# Autodesk Inventor assembly: ASY Beshkino_bio_tank
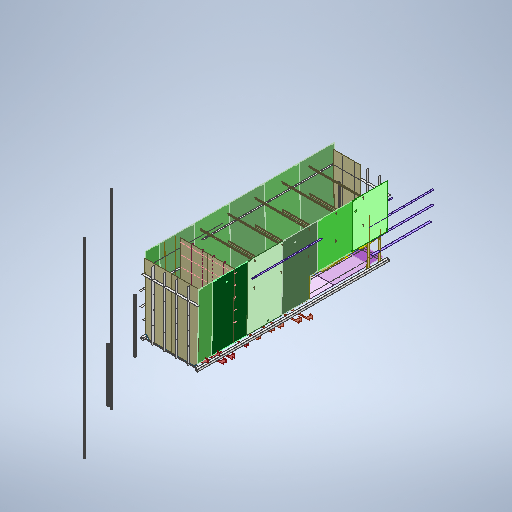
[picture p0: Inventor's stored thumbnail of the model, 512x512]
Saved by Autodesk Inventor 2025 (Build 290162010, 162A)
## iProperties
Created: 2024-07-21
Part Number: ASY Beshkino_bio_tank
Document SubType Name: Assembly
Designer: admin
Mass: 5.81287e+06 g
Surface Area: 2.77755e+06 cm^2
Volume: 3.12018e+06 cm^3
Density: 1.86299 g/cm^3
Author: admin
## Documents named in this file (40)
- C:\Users\pokla\Documents\Inventor\BSH_Beshkino_bio_tank\ASY Beshkino_bio_tank.iam
- C:\Users\pokla\Documents\Inventor\BSH_Beshkino_bio_tank\BSH 000 dim Beshkino_bio_tank.ipt
- C:\Users\pokla\Documents\Inventor\BSH_Beshkino_bio_tank\BSH 011 floor.ipt
- C:\Users\pokla\Documents\Inventor\BSH_Beshkino_bio_tank\BSH 021 rib floor.ipt
- C:\Users\pokla\Documents\Inventor\BSH_Beshkino_bio_tank\BSH 022 rib board.ipt
- C:\Users\pokla\Documents\Inventor\BSH_Beshkino_bio_tank\BSH 076 tube.ipt
- C:\Users\pokla\Documents\Inventor\BSH_Beshkino_bio_tank\BSH 061 butt end.ipt
- C:\Users\pokla\Documents\Inventor\BSH_Beshkino_bio_tank\BSH 041 board.ipt
- C:\Users\pokla\Documents\Inventor\BSH_Beshkino_bio_tank\BSH 047 board.ipt
- C:\Users\pokla\Documents\Inventor\BSH_Beshkino_bio_tank\BSH 033 stringer board 1.ipt
- C:\Users\pokla\Documents\Inventor\BSH_Beshkino_bio_tank\BSH 045 back.ipt
- C:\Users\pokla\Documents\Inventor\BSH_Beshkino_bio_tank\BSH 031 stringer floor.ipt
- C:\Users\pokla\Documents\Inventor\BSH_Beshkino_bio_tank\BSH 034 stringer board 2.ipt
- C:\Users\pokla\Documents\Inventor\BSH_Beshkino_bio_tank\BSH 035 stringer board 3.ipt
- C:\Users\pokla\Documents\Inventor\BSH_Beshkino_bio_tank\BSH 036 stringer board 4.ipt
- C:\Users\pokla\Documents\Inventor\BSH_Beshkino_bio_tank\BSH 032 stringer floor small.ipt
- C:\Users\pokla\Documents\Inventor\BSH_Beshkino_bio_tank\BSH 039 stringer butt end in.ipt
- C:\Users\pokla\Documents\Inventor\BSH_Beshkino_bio_tank\BSH 014 board cone.ipt
- C:\Users\pokla\Documents\Inventor\BSH_Beshkino_bio_tank\BSH 051 sheet in.ipt
- C:\Users\pokla\Documents\Inventor\BSH_Beshkino_bio_tank\BSH 071 amplifier in.ipt
- C:\Users\pokla\Documents\Inventor\BSH_Beshkino_bio_tank\BSH 072 amplifier in.ipt
- C:\Users\pokla\Documents\Inventor\BSH_Beshkino_bio_tank\BSH 012 floor.ipt
- C:\Users\pokla\Documents\Inventor\BSH_Beshkino_bio_tank\BSH 016 cone.ipt
- C:\Users\pokla\Documents\Inventor\BSH_Beshkino_bio_tank\BSH 013 floor.ipt
- C:\Users\pokla\Documents\Inventor\BSH_Beshkino_bio_tank\BSH 015 board cone wall.ipt
- C:\Users\pokla\Documents\Inventor\BSH_Beshkino_bio_tank\BSH 017 small detail floor.ipt
- C:\Users\pokla\Documents\Inventor\BSH_Beshkino_bio_tank\BSH 038 stringer butt end.ipt
- C:\Users\pokla\Documents\Inventor\BSH_Beshkino_bio_tank\BSH 053 sheet in.ipt
- C:\Users\pokla\Documents\Inventor\BSH_Beshkino_bio_tank\BSH 044 board.ipt
- C:\Users\pokla\Documents\Inventor\BSH_Beshkino_bio_tank\BSH 046 back.ipt
- C:\Users\pokla\Documents\Inventor\BSH_Beshkino_bio_tank\BSH 042 board.ipt
- C:\Users\pokla\Documents\Inventor\BSH_Beshkino_bio_tank\BSH 043 board.ipt
- C:\Users\pokla\Documents\Inventor\BSH_Beshkino_bio_tank\BSH 052 sheet in.ipt
- C:\Users\pokla\Documents\Inventor\BSH_Beshkino_bio_tank\BSH 023 rib butt end.ipt
- C:\Users\pokla\Documents\Inventor\BSH_Beshkino_bio_tank\BSH 037 stringer board.ipt
- C:\Users\pokla\Documents\Inventor\BSH_Beshkino_bio_tank\BSH 024 rib butt end in.ipt
- C:\Users\pokla\Documents\Inventor\BSH_Beshkino_bio_tank\BSH 077 tube.ipt
- C:\Users\pokla\Documents\Inventor\BSH_Beshkino_bio_tank\BSH 073 tube.ipt
- C:\Users\pokla\Documents\Inventor\BSH_Beshkino_bio_tank\BSH 074 tube.ipt
- C:\Users\pokla\Documents\Inventor\BSH_Beshkino_bio_tank\BSH 075 tube.ipt
## Components (114 placed, 43 different names)
1. BSH 000 dim Beshkino_bio_tank.ipt:1
2. BSH 022 rib 2.ipt:1 — Rigid:27, Rigid:28, Rigid:29, Rigid:30, Flush:114, Rigid:138
3. BSH 061 tube 1.ipt:1 — Mate:1, Rigid:1, Mate:3, Mate:119, Flush:121, Flush:122, Mate:121, Flush:123
4. BSH 061 tube 1.ipt:2 — Mate:2, Rigid:1, Mate:4, Flush:3, Flush:4, Flush:124
5. BSH 010 floor 1.ipt:2 — Rigid:5, Rigid:83, Mate:77, Flush:18, Flush:19
6. BSH 010 floor 1.ipt:3 — Rigid:5, Rigid:82
7. BSH 010 floor 1.ipt:1 — Mate:5, Mate:6, Mate:7, Flush:4, Mate:10, Flush:5, Flush:11, Rigid:82, Mate:74
8. BSH 031 nose 1.ipt:1 — Mate:10, Flush:5, Mate:11, Rigid:11, Mate:73, Mate:108
9. BSH 033 board 3.ipt:1 — Flush:11, Mate:73, Mate:74, Rigid:104
10. BSH 031 nose 1.ipt:2 — Rigid:11, Rigid:53
11. BSH 021 rib 1.ipt:1 — Mate:4, Flush:3, Mate:5, Mate:6, Rigid:9, Rigid:109, Rigid:118, Rigid:122, Mate:120
12. BSH 031 nose 1:3 — Mate:113
13. BSH 031 nose 1:4 — Rigid:53, Flush:112
14. BSH 033 board cone 3:1 — Mate:26, Rigid:57, Mate:30, Mate:80, Mate:83
15. BSH 031 nose 1:7 — Mate:26, Mate:30, Mate:84, Flush:21, Mate:94
16. BSH 031 nose 1:8 — Flush:8, Mate:40, Mate:111
17. BSH 033 board cone 3:2 — Rigid:57, Angle:1, Mate:49, Mate:50, Mate:64, Mate:71
18. BSH 043 stringer 3.ipt:1 — Rigid:29
19. BSH 042 stringer 2.ipt:1 — Rigid:28
20. BSH 041 stringer 1.ipt:1 — Rigid:27
21. BSH 041 stringer 1.ipt:2
22. BSH 042 stringer 2.ipt:2
23. BSH 043 stringer 3.ipt:2
24. BSH 044 stringer 4.ipt:2 — Rigid:127, Mate:109
25. BSH 034 board cone 4:2 — Mate:84, Rigid:108, Mate:88, Mate:89, Mate:90, Mate:91, Mate:123
26. BSH 012 floor 2:1 — Rigid:66, Mate:42, Angle:1, Mate:49, Rigid:83, Mate:72, Mate:87
27. BSH 037 cone 3:1 — Mate:42, Mate:50, Mate:90
28. BSH 033 board 3:2 — Rigid:139
29. BSH 012 floor 2:2 — Rigid:66, Rigid:67, Mate:63, Mate:78, Mate:122
30. BSH 013 floor 3:1 — Rigid:67, Mate:40, Mate:81
31. BSH 039 back 9:2 — Rigid:90, Rigid:103
32. BSH 015 board cone 5:1 — Mate:71, Mate:72, Mate:85, Mate:86
33. BSH 038 divider:1 — Mate:77, Flush:18, Flush:19
34. BSH 046 stringer 6:1 — Mate:107, Mate:108, Mate:109, Rigid:128, Rigid:129, Rigid:130, Rigid:131
35. BSH 037 cone 3:2 — Mate:63, Mate:64, Mate:91
36. BSH 044 stringer 4:3
37. BSH 044 stringer 4:4 — Mate:112
38. BSH 022 rib 2:34 — Rigid:127, Rigid:137, Mate:117, Flush:117
39. BSH 021 rib 1.ipt:2 — Rigid:9
40. BSH 037 cone 3:3 — Mate:78, Mate:80, Mate:88
41. BSH 037 cone 3:4 — Mate:81, Mate:83, Mate:89
42. BSH 035 board cone 5:1 — Rigid:107
43. BSH 035 board :1 — Rigid:90, Mate:85, Rigid:106
44. BSH 020 rib 1:5
45. BSH 020 rib 1:6
46. BSH 020 rib 1:7 — Rigid:94
47. BSH 020 rib 1:8 — Rigid:94
48. BSH 020 rib 1:9
49. BSH 020 rib 1:10
50. BSH 020 rib 1:11
51. BSH 051 back 1:1 — Rigid:103, Flush:21, Mate:96, Flush:114
52. BSH 052 board 2:1 — Rigid:104, Rigid:105
53. BSH 044 stringer 4.ipt:1 — Rigid:30
54. BSH 053 board 3:1 — Rigid:105, Rigid:106
55. BSH 054 board cone 4:1 — Rigid:107, Rigid:108, Mate:86, Mate:87
56. BSH 041 stringer floor:1 — Rigid:109, Rigid:114
57. BSH 042 stringer floor:1 — Rigid:113
58. BSH 041 stringer floor:2 — Rigid:112, Rigid:114
59. BSH 041 stringer floor:3 — Rigid:112, Rigid:113
60. BSH 041 stringer floor:4 — Rigid:118
61. BSH 042 stringer floor:2
62. BSH 041 stringer floor:5
63. BSH 041 stringer floor:6
64. BSH 041 stringer floor:7 — Rigid:122
65. BSH 042 stringer floor:3
66. BSH 041 stringer floor:8
67. BSH 041 stringer floor:9
68. BSH 041 stringer floor:10
69. BSH 041 stringer floor:11
70. BSH 041 stringer floor:12
71. BSH 023 rib 3:1 — Rigid:128
72. BSH 023 rib 3:2 — Rigid:129
73. BSH 023 rib 3:3 — Rigid:130
74. BSH 023 rib 3:4 — Rigid:131
75. BSH 046 stringer 6:2 — Flush:111, Mate:111, Mate:112
76. BSH 023 rib 3:5
77. BSH 023 rib 3:6
78. BSH 023 rib 3:7
79. BSH 023 rib 3:8
80. BSH 020 rib 1:12
81. BSH 022 rib 2:33 — Rigid:138
82. BSH 0442 stringer 42:1
83. BSH 022 rib 2:35 — Rigid:137
84. BSH 062 tube 2+:1 — Mate:119, Flush:121, Flush:122, Mate:120
85. BSH 062 tube 2+:2 — Mate:121, Flush:123, Flush:124
86. BSH 063 tube 3+:1 — Mate:122, Mate:123, Mate:124
87. BSH 064 tube 4+:1
88. BSH 065 tube 5+:1
89. BSH 064 tube 4+:2
90. BSH 065 tube 5+:2
91. BSH 032 board 2:4 — Mate:117, Flush:117, Rigid:139
92. BSH 032 board 2:5
93. BSH 032 board 2:6
94. BSH 032 board 2:7
95. BSH 032 board 2:8
96. BSH 035 divider 1:1 — Flush:22, Mate:94, Mate:96, Flush:24, Mate:97, Mate:124
97. BSH 036 divider 2:1 — Flush:22, Mate:93, Flush:24
98. BSH 035 divider 1:2
99. BSH 036 divider 2:2
100. BSH 035 divider 1:3
101. BSH 036 divider 2:3
102. BSH 035 divider 1:4
103. BSH 036 divider 2:4
104. BSH 035 divider 1:5
105. BSH 036 divider 2:5
106. BSH 045 stringer 5:1 — Mate:23, Flush:112, Mate:113, Rigid:140
107. BSH 045 stringer 5:2
108. BSH 045 stringer 5:3
109. BSH 045 stringer 5:4
110. BSH 045 stringer 5:5
111. BSH 046 stringer 6:3 — Rigid:140
112. BSH 046 stringer 6:4
113. BSH 046 stringer 6:5
114. BSH 046 stringer 6:6
## Component patterns: (5 elements, first: BSH 032 board 2:4), (5 elements, first: BSH 035 divider 1:1 + BSH 036 divider 2:1), (5 elements, first: BSH 045 stringer 5:1), (4 elements, first: BSH 046 stringer 6:3)
## Relationships (120: Mate 52, WeldJoint 49, Flush 18, Angle 1)
- Mate:1: BSH 061 tube 1.ipt:1
- Mate:2: BSH 061 tube 1.ipt:2
- Rigid:1 [WeldJoint] (-2400 mm): BSH 061 tube 1.ipt:1 ↔ BSH 061 tube 1.ipt:2
- Mate:3: BSH 061 tube 1.ipt:1
- Mate:4: BSH 061 tube 1.ipt:2 ↔ BSH 021 rib 1.ipt:1
- Flush:3: BSH 061 tube 1.ipt:2 ↔ BSH 021 rib 1.ipt:1
- Mate:5: BSH 010 floor 1.ipt:1 ↔ BSH 021 rib 1.ipt:1
- Mate:6: BSH 010 floor 1.ipt:1 ↔ BSH 021 rib 1.ipt:1
- Rigid:5 [WeldJoint]: BSH 010 floor 1.ipt:2 ↔ BSH 010 floor 1.ipt:3
- Mate:7: BSH 010 floor 1.ipt:1
- Flush:4 (100 mm): BSH 061 tube 1.ipt:2 ↔ BSH 010 floor 1.ipt:1
- Rigid:9 [WeldJoint] (-500 mm): BSH 021 rib 1.ipt:1 ↔ BSH 021 rib 1.ipt:2
- Mate:10: BSH 010 floor 1.ipt:1 ↔ BSH 031 nose 1.ipt:1
- Flush:5 (10 mm): BSH 010 floor 1.ipt:1 ↔ BSH 031 nose 1.ipt:1
- Mate:11: BSH 031 nose 1.ipt:1
- Rigid:11 [WeldJoint]: BSH 031 nose 1.ipt:1 ↔ BSH 031 nose 1.ipt:2
- Rigid:27 [WeldJoint] (2 mm): BSH 022 rib 2.ipt:1 ↔ BSH 041 stringer 1.ipt:1
- Rigid:28 [WeldJoint] (2 mm): BSH 022 rib 2.ipt:1 ↔ BSH 042 stringer 2.ipt:1
- Rigid:29 [WeldJoint] (2 mm): BSH 022 rib 2.ipt:1 ↔ BSH 043 stringer 3.ipt:1
- Rigid:30 [WeldJoint] (2 mm): BSH 022 rib 2.ipt:1 ↔ BSH 044 stringer 4.ipt:1
- Mate:23: BSH 045 stringer 5:1
- [WeldJoint]: BSH 031 nose 1:3 ↔ BSH 031 nose 1:4
- Rigid:53 [WeldJoint] (1500 mm): BSH 031 nose 1.ipt:2 ↔ BSH 031 nose 1:4
- [WeldJoint]: BSH 031 nose 1:7 ↔ BSH 031 nose 1:8
- Flush:8: BSH 031 nose 1:8
- Mate:26: BSH 033 board cone 3:1 ↔ BSH 031 nose 1:7
- Rigid:57 [WeldJoint]: BSH 033 board cone 3:1 ↔ BSH 033 board cone 3:2
- Mate:30: BSH 033 board cone 3:1 ↔ BSH 031 nose 1:7
- Flush:11: BSH 010 floor 1.ipt:1 ↔ BSH 033 board 3.ipt:1
- Rigid:66 [WeldJoint]: BSH 012 floor 2:1 ↔ BSH 012 floor 2:2
- Rigid:67 [WeldJoint]: BSH 012 floor 2:2 ↔ BSH 013 floor 3:1
- Mate:40: BSH 031 nose 1:8 ↔ BSH 013 floor 3:1
- Mate:42: BSH 012 floor 2:1 ↔ BSH 037 cone 3:1
- Angle:1 (132 deg): BSH 033 board cone 3:2 ↔ BSH 012 floor 2:1
- Mate:49: BSH 033 board cone 3:2 ↔ BSH 012 floor 2:1
- Mate:50: BSH 033 board cone 3:2 ↔ BSH 037 cone 3:1
- Mate:63: BSH 012 floor 2:2 ↔ BSH 037 cone 3:2
- Mate:64: BSH 033 board cone 3:2 ↔ BSH 037 cone 3:2
- Rigid:82 [WeldJoint]: BSH 010 floor 1.ipt:3 ↔ BSH 010 floor 1.ipt:1
- Rigid:83 [WeldJoint]: BSH 010 floor 1.ipt:2 ↔ BSH 012 floor 2:1
- Mate:71: BSH 033 board cone 3:2 ↔ BSH 015 board cone 5:1
- Mate:72: BSH 012 floor 2:1 ↔ BSH 015 board cone 5:1
- Mate:73: BSH 031 nose 1.ipt:1 ↔ BSH 033 board 3.ipt:1
- Mate:74: BSH 010 floor 1.ipt:1 ↔ BSH 033 board 3.ipt:1
- Mate:77: BSH 010 floor 1.ipt:2 ↔ BSH 038 divider:1
- Flush:18: BSH 010 floor 1.ipt:2 ↔ BSH 038 divider:1
- Flush:19: BSH 010 floor 1.ipt:2 ↔ BSH 038 divider:1
- Mate:78: BSH 012 floor 2:2 ↔ BSH 037 cone 3:3
- Mate:80: BSH 033 board cone 3:1 ↔ BSH 037 cone 3:3
- Mate:81: BSH 013 floor 3:1 ↔ BSH 037 cone 3:4
- Mate:83: BSH 033 board cone 3:1 ↔ BSH 037 cone 3:4
- Mate:84: BSH 031 nose 1:7 ↔ BSH 034 board cone 4:2
- Rigid:90 [WeldJoint]: BSH 039 back 9:2 ↔ BSH 035 board :1
- Mate:85: BSH 015 board cone 5:1 ↔ BSH 035 board :1
- Rigid:94 [WeldJoint] (500 mm): BSH 020 rib 1:7 ↔ BSH 020 rib 1:8
- Rigid:103 [WeldJoint]: BSH 039 back 9:2 ↔ BSH 051 back 1:1
- Rigid:104 [WeldJoint]: BSH 033 board 3.ipt:1 ↔ BSH 052 board 2:1
- Rigid:105 [WeldJoint]: BSH 052 board 2:1 ↔ BSH 053 board 3:1
- Rigid:106 [WeldJoint]: BSH 035 board :1 ↔ BSH 053 board 3:1
- Flush:21 (10 mm): BSH 031 nose 1:7 ↔ BSH 051 back 1:1
- Rigid:107 [WeldJoint]: BSH 035 board cone 5:1 ↔ BSH 054 board cone 4:1
- Rigid:108 [WeldJoint]: BSH 034 board cone 4:2 ↔ BSH 054 board cone 4:1
- Mate:86: BSH 015 board cone 5:1 ↔ BSH 054 board cone 4:1
- Mate:87: BSH 012 floor 2:1 ↔ BSH 054 board cone 4:1
- Mate:88: BSH 034 board cone 4:2 ↔ BSH 037 cone 3:3
- Mate:89: BSH 034 board cone 4:2 ↔ BSH 037 cone 3:4
- Mate:90: BSH 034 board cone 4:2 ↔ BSH 037 cone 3:1
- Mate:91: BSH 034 board cone 4:2 ↔ BSH 037 cone 3:2
- Flush:22: BSH 035 divider 1:1 ↔ BSH 036 divider 2:1
- Mate:93: BSH 036 divider 2:1
- Mate:94 (1000 mm): BSH 031 nose 1:7 ↔ BSH 035 divider 1:1
- Rigid:109 [WeldJoint] (2 mm): BSH 021 rib 1.ipt:1 ↔ BSH 041 stringer floor:1
- Rigid:112 [WeldJoint] (-20 mm): BSH 041 stringer floor:2 ↔ BSH 041 stringer floor:3
- Rigid:113 [WeldJoint] (-250.2 mm): BSH 042 stringer floor:1 ↔ BSH 041 stringer floor:3
- Rigid:114 [WeldJoint] (-20 mm): BSH 041 stringer floor:1 ↔ BSH 041 stringer floor:2
- [WeldJoint] (-20 mm): BSH 041 stringer floor:5 ↔ BSH 041 stringer floor:6
- [WeldJoint] (-250.2 mm): BSH 042 stringer floor:2 ↔ BSH 041 stringer floor:6
- [WeldJoint] (-20 mm): BSH 041 stringer floor:4 ↔ BSH 041 stringer floor:5
- Rigid:118 [WeldJoint] (2 mm): BSH 021 rib 1.ipt:1 ↔ BSH 041 stringer floor:4
- [WeldJoint] (-20 mm): BSH 041 stringer floor:8 ↔ BSH 041 stringer floor:9
- [WeldJoint] (-250.2 mm): BSH 042 stringer floor:3 ↔ BSH 041 stringer floor:9
- [WeldJoint] (-20 mm): BSH 041 stringer floor:7 ↔ BSH 041 stringer floor:8
- Rigid:122 [WeldJoint] (2 mm): BSH 021 rib 1.ipt:1 ↔ BSH 041 stringer floor:7
- Mate:96 (100 mm): BSH 051 back 1:1 ↔ BSH 035 divider 1:1
- Flush:24 (1000 mm): BSH 035 divider 1:1 ↔ BSH 036 divider 2:1
- Mate:97: BSH 035 divider 1:1
- Rigid:127 [WeldJoint] (2 mm): BSH 044 stringer 4.ipt:2 ↔ BSH 022 rib 2:34
- Mate:107: BSH 046 stringer 6:1
- Mate:108: BSH 031 nose 1.ipt:1 ↔ BSH 046 stringer 6:1
- Mate:109: BSH 044 stringer 4.ipt:2 ↔ BSH 046 stringer 6:1
- Rigid:128 [WeldJoint] (2 mm): BSH 046 stringer 6:1 ↔ BSH 023 rib 3:1
- Rigid:129 [WeldJoint] (2 mm): BSH 046 stringer 6:1 ↔ BSH 023 rib 3:2
- Rigid:130 [WeldJoint] (2 mm): BSH 046 stringer 6:1 ↔ BSH 023 rib 3:3
- Rigid:131 [WeldJoint] (2 mm): BSH 046 stringer 6:1 ↔ BSH 023 rib 3:4
- [WeldJoint] (2 mm): BSH 046 stringer 6:2 ↔ BSH 023 rib 3:5
- [WeldJoint] (2 mm): BSH 046 stringer 6:2 ↔ BSH 023 rib 3:6
- [WeldJoint] (2 mm): BSH 046 stringer 6:2 ↔ BSH 023 rib 3:7
- [WeldJoint] (2 mm): BSH 046 stringer 6:2 ↔ BSH 023 rib 3:8
- Flush:111: BSH 046 stringer 6:2
- Mate:111: BSH 031 nose 1:8 ↔ BSH 046 stringer 6:2
- Mate:112: BSH 044 stringer 4:4 ↔ BSH 046 stringer 6:2
- Flush:112 (171.5 mm): BSH 031 nose 1:4 ↔ BSH 045 stringer 5:1
- Mate:113: BSH 031 nose 1:3 ↔ BSH 045 stringer 5:1
- Flush:114 (246.5 mm): BSH 022 rib 2.ipt:1 ↔ BSH 051 back 1:1
- Rigid:137 [WeldJoint] (-436 mm): BSH 022 rib 2:34 ↔ BSH 022 rib 2:35
- Mate:117: BSH 022 rib 2:34 ↔ BSH 032 board 2:4
- Flush:117 (-218 mm): BSH 022 rib 2:34 ↔ BSH 032 board 2:4
- Rigid:138 [WeldJoint] (-493 mm): BSH 022 rib 2.ipt:1 ↔ BSH 022 rib 2:33
- Rigid:139 [WeldJoint]: BSH 033 board 3:2 ↔ BSH 032 board 2:4
- Rigid:140 [WeldJoint] (2 mm): BSH 045 stringer 5:1 ↔ BSH 046 stringer 6:3
- Mate:119: BSH 061 tube 1.ipt:1 ↔ BSH 062 tube 2+:1
- Flush:121: BSH 061 tube 1.ipt:1 ↔ BSH 062 tube 2+:1
- Flush:122 (90 mm): BSH 061 tube 1.ipt:1 ↔ BSH 062 tube 2+:1
- Mate:120 (248.5 mm): BSH 021 rib 1.ipt:1 ↔ BSH 062 tube 2+:1
- Mate:121: BSH 061 tube 1.ipt:1 ↔ BSH 062 tube 2+:2
- Flush:123: BSH 061 tube 1.ipt:1 ↔ BSH 062 tube 2+:2
- Flush:124 (-90 mm): BSH 061 tube 1.ipt:2 ↔ BSH 062 tube 2+:2
- Mate:122: BSH 012 floor 2:2 ↔ BSH 063 tube 3+:1
- Mate:123: BSH 034 board cone 4:2 ↔ BSH 063 tube 3+:1
- Mate:124: BSH 063 tube 3+:1 ↔ BSH 035 divider 1:1
## Named parameters: d118_d31 = 0 mm, d124_d31 = 0 mm, d324_d323 = -20 mm, d325_d318 = -20 mm, d326_d319 = -250.2 mm, d328_d323 = -20 mm, d329_d318 = -20 mm, d330_d319 = -250.2 mm, d381_d380 = 2 mm, d382_d377 = 2 mm, d383_d378 = 2 mm, d384_d379 = 2 mm
